# Autodesk Inventor assembly: Assembly2
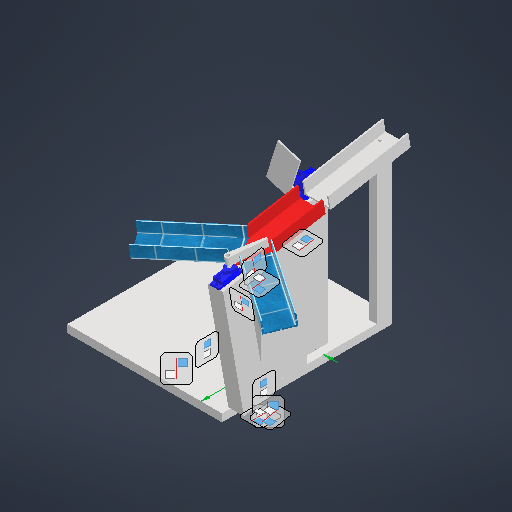
[picture p0: Inventor's stored thumbnail of the model, 512x512]
Saved by Autodesk Inventor 2026.2 (Build 302298000, 298)
## iProperties
Created: 2026-02-23
Part Number: Assembly2
Document SubType Name: Assembly
Designer: danda
Author: danda
## Documents named in this file (14)
- C:\Users\danda\OneDrive\Desktop\Basics Of Mecha\Project\Assembly2.iam
- C:\Users\danda\OneDrive\Desktop\Basics Of Mecha\Project\stand.ipt
- C:\Users\danda\OneDrive\Desktop\Basics Of Mecha\Project\stand2.ipt
- C:\Users\danda\OneDrive\Desktop\Basics Of Mecha\Project\inslide.ipt
- C:\Users\danda\OneDrive\Desktop\Basics Of Mecha\Project\base.ipt
- C:\Users\danda\OneDrive\Desktop\Basics Of Mecha\Project\Towerpro Micro Servo 9g\Towerpro Micro Servo 9g\Towerpro Micro Servo 9g.ipt
- C:\Users\danda\OneDrive\Desktop\Basics Of Mecha\Project\motorstand1.ipt
- C:\Users\danda\OneDrive\Desktop\Basics Of Mecha\Project\gate.ipt
- C:\Users\danda\OneDrive\Desktop\Basics Of Mecha\Project\middleslide.ipt
- C:\Users\danda\OneDrive\Desktop\Basics Of Mecha\Project\motorstand2.ipt
- C:\Users\danda\OneDrive\Desktop\Basics Of Mecha\Project\gate2.ipt
- C:\Users\danda\OneDrive\Desktop\Basics Of Mecha\Project\wedge.ipt
- C:\Users\danda\OneDrive\Desktop\Basics Of Mecha\Project\outslide.ipt
- C:\Users\danda\OneDrive\Desktop\Basics Of Mecha\Project\outslideleft.ipt
## Components (14 placed, 13 different names)
1. stand:1 — Mate:5, Flush:8, Flush:9, Mate:30, Mate:33, Flush:14, Mate:34
2. stand2:1 — Mate:4, Flush:1, Flush:7, Mate:17, Mate:18, Mate:30, Mate:31, Mate:32, Flush:13
3. inslide:1 — Flush:8, Mate:17, Mate:18, Mate:31, Mate:32, Flush:13
4. base:1 — Mate:3, Mate:4, Flush:1, Mate:5, Mate:9, Mate:14, Mate:15, Flush:7, Mate:26, Flush:10, Mate:29, Flush:12, Flush:15
5. Towerpro Micro Servo 9g:1 — Mate:11, Mate:12, Mate:13, Insert:1
6. motorstand1:1 — Mate:9, Mate:11, Mate:12, Mate:13, Flush:12, Flush:15
7. gate:1 — Insert:1
8. middleslide:1 — Flush:9, Mate:33, Flush:14, Mate:34, Flush:16, Mate:35, Mate:36, Mate:37, Flush:17, Mate:38
9. motorstand2:1 — Mate:21, Mate:22, Mate:23, Mate:27, Flush:11, Mate:28
10. Towerpro Micro Servo 9g:2 — Mate:21, Mate:22, Mate:23, Insert:2, Rotational:1
11. gate2:1 — Insert:2, Rotational:1
12. wedge:1 — Mate:26, Flush:10, Mate:27, Flush:11, Mate:28, Mate:29
13. outslide:1 — Flush:16, Mate:35, Mate:36
14. outslideleft:1 — Mate:37, Flush:17, Mate:38
## Relationships (42: Mate 27, Flush 12, Insert 2, RevoluteJoint 1)
- Mate:3: base:1
- Mate:4: stand2:1 ↔ base:1
- Flush:1: stand2:1 ↔ base:1
- Mate:5: stand:1 ↔ base:1
- Mate:9: base:1 ↔ motorstand1:1
- Mate:11: Towerpro Micro Servo 9g:1 ↔ motorstand1:1
- Mate:12: Towerpro Micro Servo 9g:1 ↔ motorstand1:1
- Mate:13: Towerpro Micro Servo 9g:1 ↔ motorstand1:1
- Insert:1: Towerpro Micro Servo 9g:1 ↔ gate:1
- Mate:14: base:1
- Mate:15: base:1
- Flush:7: stand2:1 ↔ base:1
- Flush:8: stand:1 ↔ inslide:1
- Mate:17: stand2:1 ↔ inslide:1
- Mate:18: stand2:1 ↔ inslide:1
- Flush:9: stand:1 ↔ middleslide:1
- Mate:21: motorstand2:1 ↔ Towerpro Micro Servo 9g:2
- Mate:22: motorstand2:1 ↔ Towerpro Micro Servo 9g:2
- Mate:23: motorstand2:1 ↔ Towerpro Micro Servo 9g:2
- Mate:26: base:1 ↔ wedge:1
- Flush:10: base:1 ↔ wedge:1
- Mate:27: motorstand2:1 ↔ wedge:1
- Flush:11: motorstand2:1 ↔ wedge:1
- Mate:28: motorstand2:1 ↔ wedge:1
- Mate:29 (11 mm): base:1 ↔ wedge:1
- Insert:2: Towerpro Micro Servo 9g:2 ↔ gate2:1
- Flush:12 (119.38 mm): base:1 ↔ motorstand1:1
- Mate:30 (90 mm): stand:1 ↔ stand2:1
- Mate:31: stand2:1 ↔ inslide:1
- Mate:32: stand2:1 ↔ inslide:1
- Flush:13: stand2:1 ↔ inslide:1
- Mate:33: stand:1 ↔ middleslide:1
- Flush:14: stand:1 ↔ middleslide:1
- Mate:34: stand:1 ↔ middleslide:1
- Flush:15 (10.16 mm): base:1 ↔ motorstand1:1
- Flush:16: middleslide:1 ↔ outslide:1
- Mate:35: middleslide:1 ↔ outslide:1
- Mate:36: middleslide:1 ↔ outslide:1
- Mate:37: middleslide:1 ↔ outslideleft:1
- Flush:17: middleslide:1 ↔ outslideleft:1
- Mate:38: middleslide:1 ↔ outslideleft:1
- Rotational:1 [RevoluteJoint]: Towerpro Micro Servo 9g:2 ↔ gate2:1
## Named parameters: Finish1_Area = 236.408, Finish2_Area = 72.9614
note: some values were not read from the file. Shown as the stored number, unit unknown: "Finish1_Area", "Finish2_Area".
